# Autodesk Inventor assembly: Fan_Mount_Assembly
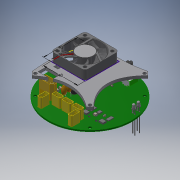
[picture p0: Inventor's stored thumbnail of the model, 180x180]
Saved by Autodesk Inventor 2019 (Build 230136000, 136)
## iProperties
Created: 2019-03-15
Part Number: Fan_Mount_Assembly
Document SubType Name: Assembly
Designer: Jorian Bruslind
Author: Jorian Bruslind
## Documents named in this file (4)
- C:\Users\Jorian Bruslind\Documents\GitHub\PersonalProjects\Inventor Projects\ROV_Models\Fan_Mount_Assembly.iam
- C:\Users\Jorian Bruslind\Documents\GitHub\PersonalProjects\Inventor Projects\ROV_Models\Fan_Mount.ipt
- C:\Users\Jorian Bruslind\Downloads\LM5085 Bucker convert\ExportSTEP\LM5085.iam
- E:\Downloads\40mm-dc-fan-1.snapshot.7\40x40x10 DC Fan.ipt
## Components (3 placed, 3 different names)
1. Fan_Mount:1 — Mate:1, Mate:2, Mate:3, Mate:4, Mate:5
2. LM5085:1 [sub-assembly] — Mate:1, Mate:2, Mate:3
3. 40x40x10 DC Fan:1 — Mate:4, Mate:5
## Relationships (5: Mate 5)
- Mate:1 (20 mm): Fan_Mount:1 ↔ LM5085:1
- Mate:2: Fan_Mount:1 ↔ LM5085:1
- Mate:3: Fan_Mount:1 ↔ LM5085:1
- Mate:4: Fan_Mount:1 ↔ 40x40x10 DC Fan:1
- Mate:5: Fan_Mount:1 ↔ 40x40x10 DC Fan:1
